# Autodesk Inventor assembly: Servo_DS3218MG
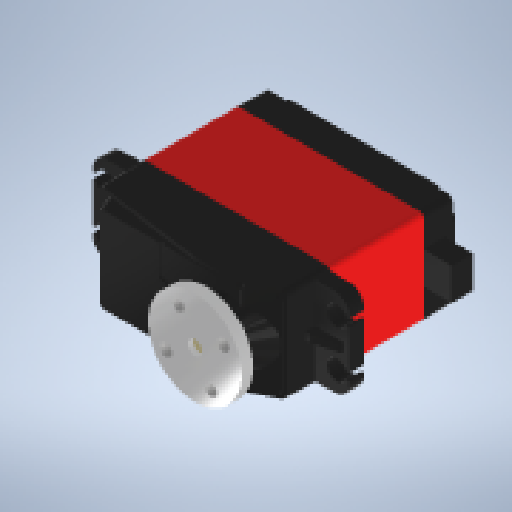
[picture p0: Inventor's stored thumbnail of the model, 512x512]
Saved by Autodesk Inventor 2023 (Build 270158000, 158)
## iProperties
Created: 2020-11-09
Part Number: Servo_DS3218MG
Document SubType Name: Assembly
Designer: Hagihara Yuya
Author: Hagihara Yuya
## Documents named in this file (3)
- C:\Users\田之上巧太\Desktop\Basic_Parts\BasicParts\ServoMotor\Servo_DS3218MG\@Servo_DS3218MG.iam
- C:\Users\田之上巧太\Desktop\Basic_Parts\BasicParts\ServoMotor\Servo_DS3218MG\DS3218MG.ipt
- C:\Users\田之上巧太\Desktop\Basic_Parts\BasicParts\ServoMotor\Servo_DS3218MG\サーボモータ25kgcmサーボホーン1.ipt
## Components (2 placed, 2 different names)
1. DS3218MG:1 — 回転:1
2. サーボモータ25kgcmサーボホーン1:1 — 回転:1
## Relationships (1: RevoluteJoint 1)
- 回転:1 [RevoluteJoint]: DS3218MG:1 ↔ サーボモータ25kgcmサーボホーン1:1
